# Autodesk Inventor assembly: Сборка4
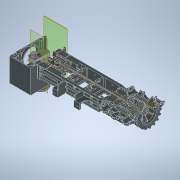
[picture p0: Inventor's stored thumbnail of the model, 180x180]
Saved by Autodesk Inventor 2021 (Build 250183000, 183)
## iProperties
Created: 2020-11-22
Part Number: Сборка4
Document SubType Name: Assembly
Designer: Тимоха
Author: Тимоха
## Documents named in this file (66)
- C:\Users\Тимоха\Desktop\КР Компрессор\compressor\Сборка4.iam
- C:\Users\Тимоха\Desktop\КР Компрессор\compressor\Верхняя часть поршня.ipt
- C:\Users\Тимоха\Desktop\КР Компрессор\compressor\Втулка.ipt
- C:\Users\Тимоха\Desktop\КР Компрессор\compressor\Гайка шток-поршень.ipt
- C:\Users\Тимоха\Desktop\КР Компрессор\compressor\Дроссельное кольцо.ipt
- C:\Users\Тимоха\Desktop\КР Компрессор\compressor\Клапан1.iam
- C:\Users\Тимоха\Desktop\КР Компрессор\compressor\Кольцо поршень-шток верх.ipt
- C:\Users\Тимоха\Desktop\КР Компрессор\compressor\Кольцо поршень-шток низ.ipt
- C:\Users\Тимоха\Desktop\КР Компрессор\compressor\Кольцо поршня.ipt
- C:\Users\Тимоха\Desktop\КР Компрессор\compressor\Кольцо сальника.ipt
- C:\Users\Тимоха\Desktop\КР Компрессор\compressor\Корпус дросселя.ipt
- C:\Users\Тимоха\Desktop\КР Компрессор\compressor\Корпус сальника.ipt
- C:\Users\Тимоха\Desktop\КР Компрессор\compressor\Крышка сальников.ipt
- C:\Users\Тимоха\Desktop\КР Компрессор\compressor\Крышка стакана.ipt
- C:\Users\Тимоха\Desktop\КР Компрессор\compressor\Крышка цилиндра 1.ipt
- C:\Users\Тимоха\Desktop\КР Компрессор\compressor\Крышка цилиндра 2.ipt
- C:\Users\Тимоха\Desktop\КР Компрессор\compressor\Нижняя часть поршня.ipt
- C:\Users\Тимоха\Desktop\КР Компрессор\compressor\Опорное кольцо.ipt
- C:\Users\Тимоха\Desktop\КР Компрессор\compressor\Прокладка клапана.ipt
- C:\Users\Тимоха\Desktop\КР Компрессор\compressor\Пружина дросселя.ipt
- C:\Users\Тимоха\Desktop\КР Компрессор\compressor\Пружина сальника.ipt
- C:\Users\Тимоха\Desktop\КР Компрессор\compressor\Стакан1.ipt
- C:\Users\Тимоха\Desktop\КР Компрессор\compressor\Цилиндр2.ipt
- C:\Users\Тимоха\Desktop\КР Компрессор\compressor\Шток.ipt
- C:\Users\Тимоха\Documents\Inventor\Content Center Files\R2021\ru-RU\Stud GOST 22034-76\Шпилька M20-6g×50 ГОСТ 22034-76.ipt
- C:\Users\Тимоха\Documents\Inventor\Content Center Files\R2021\ru-RU\GOST 10450-78\Шайба 21 ГОСТ 10450-78.ipt
- C:\Users\Тимоха\Documents\Inventor\Content Center Files\R2021\ru-RU\GOST 15521-70\Гайка M20-6H ГОСТ 15521-70.ipt
- C:\Users\Тимоха\Documents\Inventor\Content Center Files\R2021\ru-RU\GOST 11371-78  A\Шайба 24 ГОСТ 11371-78.ipt
- C:\Users\Тимоха\Documents\Inventor\Content Center Files\R2021\ru-RU\Stud GOST 22038-76\Шпилька M24-6g×70 ГОСТ 22038-76.ipt
- C:\Users\Тимоха\Documents\Inventor\Content Center Files\R2021\ru-RU\Nut GOST 15524-70\Гайка M24-6H ГОСТ 15524-70.ipt
- C:\Users\Тимоха\Documents\Inventor\Content Center Files\R2021\ru-RU\Bolt GOST R 50274-92\Болт M8-6g×20-F ГОСТ Р 50274-92.ipt
- C:\Users\Тимоха\Desktop\КР Компрессор\compressor\Деталь5.ipt
- C:\Users\Тимоха\Desktop\КР Компрессор\compressor\Деталь6.ipt
- C:\Users\Тимоха\Desktop\КР Компрессор\compressor\Прокладка воды зад.ipt
- C:\Users\Тимоха\Desktop\КР Компрессор\compressor\Крышка воды зад.ipt
- C:\Users\Тимоха\Documents\Inventor\Content Center Files\R2021\ru-RU\GOST 15521-70\Гайка M10-6H ГОСТ 15521-70.ipt
- C:\Users\Тимоха\Documents\Inventor\Content Center Files\R2021\ru-RU\Stud GOST 22034-76\Шпилька M10-6g×45 ГОСТ 22034-76.ipt
- C:\Users\Тимоха\Documents\Inventor\Content Center Files\R2021\ru-RU\Washer GOST 9065-75\Шайба 12 ГОСТ 9065-75.ipt
- C:\Users\Тимоха\Desktop\КР Компрессор\compressor\Фонарь.ipt
- C:\Users\Тимоха\Documents\Inventor\Content Center Files\R2021\ru-RU\Stud GOST 22038-76\Шпилька M20-6g×80 ГОСТ 22038-76.ipt
- C:\Users\Тимоха\Documents\Inventor\Content Center Files\R2021\ru-RU\GOST 6402-70\Шайба  22 L ГОСТ 6402-70.ipt
- C:\Users\Тимоха\Documents\Inventor\Content Center Files\R2021\ru-RU\Nut GOST ISO 8673-2014\Копия Копия гайки M20x1,5-6H ГОСТ 5915-70.ipt
- C:\Users\Тимоха\Desktop\КР Компрессор\compressor\Корпус сальника перегородка 1.ipt
- C:\Users\Тимоха\Desktop\КР Компрессор\compressor\Крышка перегородки11.ipt
- C:\Users\Тимоха\Desktop\КР Компрессор\compressor\Крышка перегородки12.ipt
- C:\Users\Тимоха\Desktop\КР Компрессор\compressor\Придав перегородки1.ipt
- C:\Users\Тимоха\Desktop\КР Компрессор\compressor\Корпус маслосъемника.ipt
- C:\Users\Тимоха\Desktop\КР Компрессор\compressor\Крышка перегородки21.ipt
- C:\Users\Тимоха\Desktop\КР Компрессор\compressor\Крышка перегородки22.ipt
- C:\Users\Тимоха\Desktop\КР Компрессор\compressor\Маслосъемная пружина.ipt
- C:\Users\Тимоха\Desktop\КР Компрессор\compressor\Маслосъемное кольцо.ipt
- C:\Users\Тимоха\Documents\Inventor\Content Center Files\R2021\ru-RU\GOST 11738-84\Винт M10-6gx20 ГОСТ 11738-84.ipt
- C:\Users\Тимоха\Documents\Inventor\Content Center Files\R2021\ru-RU\GOST 11371-78  A\Шайба 12 ГОСТ 11371-78.ipt
- C:\Users\Тимоха\Documents\Inventor\Content Center Files\R2021\ru-RU\GOST 11738-84\Винт M10-6gx25 ГОСТ 11738-84.ipt
- C:\Users\Тимоха\Desktop\КР Компрессор\compressor\Крейцкопфф.iam
- C:\Users\Тимоха\Desktop\КР Компрессор\compressor\Вал.ipt
- C:\Users\Тимоха\Desktop\КР Компрессор\compressor\Крышка фонаря 1.ipt
- C:\Users\Тимоха\Desktop\КР Компрессор\compressor\Крышка фонаря 2.ipt
- C:\Users\Тимоха\Desktop\КР Компрессор\compressor\Крышка коренного подшипника1.ipt
- C:\Users\Тимоха\Desktop\КР Компрессор\compressor\Картер.ipt
- C:\Users\Тимоха\Desktop\КР Компрессор\compressor\Балка.ipt
- C:\Users\Тимоха\Desktop\КР Компрессор\compressor\Крышка стенки картера низ.ipt
- C:\Users\Тимоха\Desktop\КР Компрессор\compressor\Нижняя часть коренного подшипника.ipt
- C:\Users\Тимоха\Desktop\КР Компрессор\compressor\Крышка стенки картера верх.ipt
- C:\Users\Тимоха\Desktop\КР Компрессор\compressor\Крышка картера 1.ipt
- C:\Users\Тимоха\Desktop\КР Компрессор\compressor\Крышка картера 3.ipt
## Components (455 placed, 65 different names)
1. Втулка:1 — Жесткий:9, Жесткий:12
2. Дроссельное кольцо:1 — Жесткий:21, Жесткий:22
3. Клапан1:1 [sub-assembly] — Жесткий:11, С поворотом:4
4. Корпус дросселя:1 — Жесткий:22, С поворотом:6
5. Крышка сальников:1 — Жесткий:72, Жесткий:73, Жесткий:143
6. Крышка стакана:1 — С поворотом:5
7. Крышка цилиндра 1:1 — Жесткий:12, С поворотом:9, Жесткий:198, Угол:1, Угол:2, Угол:3
8. Крышка цилиндра 2:1 — Жесткий:13, С поворотом:6, Жесткий:79, Жесткий:142, Жесткий:145, С поворотом:16
9. Прокладка клапана:1 — Жесткий:10, Жесткий:11
10. Пружина дросселя:1 — Жесткий:21
11. Стакан1:1 — С поворотом:4, С поворотом:5
12. Цилиндр2:1 — Жесткий:9, Жесткий:10, Жесткий:13, Жесткий:74, Жесткий:76, Жесткий:80, Заподлицо:1, Заподлицо:2, Заподлицо:5, Заподлицо:6
13. Кольцо сальника:4
14. Корпус сальника:2 — Жесткий:65
15. Пружина сальника:4
16. Кольцо сальника:5
17. Пружина сальника:5
18. Кольцо сальника:6
19. Пружина сальника:6
20. Кольцо сальника:7
21. Корпус сальника:3 — Жесткий:69, Жесткий:73
22. Пружина сальника:7
23. Кольцо сальника:8
24. Пружина сальника:8
25. Кольцо сальника:9
26. Пружина сальника:9
27. Кольцо сальника:10
28. Корпус сальника:4 — Жесткий:66
29. Пружина сальника:10
30. Кольцо сальника:11
31. Пружина сальника:11
32. Кольцо сальника:12
33. Пружина сальника:12
34. Кольцо сальника:13
35. Корпус сальника:5 — Жесткий:68
36. Пружина сальника:13
37. Кольцо сальника:14
38. Пружина сальника:14
39. Кольцо сальника:15
40. Пружина сальника:15
41. Кольцо сальника:16
42. Корпус сальника:6 — Жесткий:68, Жесткий:69
43. Пружина сальника:16
44. Кольцо сальника:17
45. Пружина сальника:17
46. Кольцо сальника:18
47. Пружина сальника:18
48. Кольцо сальника:19
49. Корпус сальника:7 — Жесткий:65, Жесткий:66
50. Пружина сальника:19
51. Кольцо сальника:20
52. Пружина сальника:20
53. Кольцо сальника:21
54. Пружина сальника:21
55. Кольцо сальника:22 — Жесткий:70, Жесткий:140
56. Кольцо сальника:23 — Жесткий:70, Жесткий:71, Жесткий:139
57. Кольцо сальника:24 — Жесткий:71, Жесткий:72, Жесткий:141
58. Болт ГОСТ Р 50274-92 M8-6g×20-F:2 — Жесткий:82
59. Болт ГОСТ Р 50274-92 M8-6g×20-F:3 — Жесткий:81
60. Деталь5:1 — Заподлицо:1, Заподлицо:2, Заподлицо:3, Заподлицо:4
61. Деталь6:1 — Заподлицо:3, Заподлицо:4, Жесткий:81, Жесткий:82, С поворотом:10, С поворотом:11, С поворотом:12, С поворотом:13, С поворотом:14, Жесткий:83, Жесткий:84, Жесткий:85, Жесткий:86, Жесткий:87, Жесткий:88, Жесткий:89, Жесткий:90, Жесткий:91, Жесткий:92, Жесткий:93, Жесткий:94, Жесткий:95, Жесткий:96, Жесткий:97, Жесткий:98, Жесткий:99, Жесткий:100, Жесткий:101, Жесткий:102, Жесткий:103, Жесткий:104, Жесткий:105, Жесткий:106, Жесткий:107
62. Прокладка воды зад:1 — Заподлицо:5, Заподлицо:6, Заподлицо:7, Заподлицо:8
63. Крышка воды зад:1 — Заподлицо:7, Заподлицо:8, С поворотом:15, Жесткий:108, Жесткий:109, Жесткий:110, Жесткий:111, Жесткий:112, Жесткий:113, Жесткий:114, Жесткий:115, Жесткий:116, Жесткий:117, Жесткий:118, Жесткий:119, Жесткий:120, Жесткий:121, Жесткий:122, Жесткий:123, Жесткий:124, Жесткий:125, Жесткий:126, Жесткий:127, Жесткий:128, Жесткий:129, Жесткий:130, Жесткий:131, Жесткий:132, Жесткий:133, Жесткий:134, Жесткий:135, Жесткий:136, Жесткий:137, Жесткий:138
64. Болт ГОСТ Р 50274-92 M8-6g×20-F:33 — С поворотом:14
65. Болт ГОСТ Р 50274-92 M8-6g×20-F:34 — Жесткий:85
66. Болт ГОСТ Р 50274-92 M8-6g×20-F:35 — С поворотом:11
67. Болт ГОСТ Р 50274-92 M8-6g×20-F:36 — С поворотом:10
68. Болт ГОСТ Р 50274-92 M8-6g×20-F:37 — Жесткий:83
69. Болт ГОСТ Р 50274-92 M8-6g×20-F:38 — Жесткий:84
70. Болт ГОСТ Р 50274-92 M8-6g×20-F:39 — С поворотом:12
71. Болт ГОСТ Р 50274-92 M8-6g×20-F:40 — С поворотом:13
72. Болт ГОСТ Р 50274-92 M8-6g×20-F:41 — Жесткий:91
73. Болт ГОСТ Р 50274-92 M8-6g×20-F:42 — Жесткий:90
74. Болт ГОСТ Р 50274-92 M8-6g×20-F:43 — Жесткий:87
75. Болт ГОСТ Р 50274-92 M8-6g×20-F:44 — Жесткий:86
76. Болт ГОСТ Р 50274-92 M8-6g×20-F:45 — Жесткий:89
77. Болт ГОСТ Р 50274-92 M8-6g×20-F:46 — Жесткий:93
78. Болт ГОСТ Р 50274-92 M8-6g×20-F:47 — Жесткий:88
79. Болт ГОСТ Р 50274-92 M8-6g×20-F:48 — Жесткий:92
80. Болт ГОСТ Р 50274-92 M8-6g×20-F:49 — Жесткий:99
81. Болт ГОСТ Р 50274-92 M8-6g×20-F:50 — Жесткий:98
82. Болт ГОСТ Р 50274-92 M8-6g×20-F:51 — Жесткий:97
83. Болт ГОСТ Р 50274-92 M8-6g×20-F:52 — Жесткий:94
84. Болт ГОСТ Р 50274-92 M8-6g×20-F:53 — Жесткий:95
85. Болт ГОСТ Р 50274-92 M8-6g×20-F:54 — Жесткий:102
86. Болт ГОСТ Р 50274-92 M8-6g×20-F:55 — Жесткий:100
87. Болт ГОСТ Р 50274-92 M8-6g×20-F:56 — Жесткий:101
88. Болт ГОСТ Р 50274-92 M8-6g×20-F:58 — Жесткий:106
89. Болт ГОСТ Р 50274-92 M8-6g×20-F:59 — Жесткий:104
90. Болт ГОСТ Р 50274-92 M8-6g×20-F:60 — Жесткий:96
91. Болт ГОСТ Р 50274-92 M8-6g×20-F:61 — Жесткий:107
92. Болт ГОСТ Р 50274-92 M8-6g×20-F:63 — Жесткий:103
93. Болт ГОСТ Р 50274-92 M8-6g×20-F:64 — Жесткий:105
94. Болт ГОСТ Р 50274-92 M8-6g×20-F:68 — С поворотом:15
95. Болт ГОСТ Р 50274-92 M8-6g×20-F:97 — Жесткий:108
96. Болт ГОСТ Р 50274-92 M8-6g×20-F:98 — Жесткий:110
97. Болт ГОСТ Р 50274-92 M8-6g×20-F:99 — Жесткий:109
98. Болт ГОСТ Р 50274-92 M8-6g×20-F:100 — Жесткий:111
99. Болт ГОСТ Р 50274-92 M8-6g×20-F:101 — Жесткий:113
100. Болт ГОСТ Р 50274-92 M8-6g×20-F:102 — Жесткий:112
101. Болт ГОСТ Р 50274-92 M8-6g×20-F:103 — Жесткий:114
102. Болт ГОСТ Р 50274-92 M8-6g×20-F:104 — Жесткий:115
103. Болт ГОСТ Р 50274-92 M8-6g×20-F:105 — Жесткий:116
104. Болт ГОСТ Р 50274-92 M8-6g×20-F:106 — Жесткий:118
105. Болт ГОСТ Р 50274-92 M8-6g×20-F:107 — Жесткий:130
106. Болт ГОСТ Р 50274-92 M8-6g×20-F:108 — Жесткий:134
107. Болт ГОСТ Р 50274-92 M8-6g×20-F:109 — Жесткий:133
108. Болт ГОСТ Р 50274-92 M8-6g×20-F:110 — Жесткий:131
109. Болт ГОСТ Р 50274-92 M8-6g×20-F:111 — Жесткий:135
110. Болт ГОСТ Р 50274-92 M8-6g×20-F:112 — Жесткий:132
111. Болт ГОСТ Р 50274-92 M8-6g×20-F:117 — Жесткий:117
112. Болт ГОСТ Р 50274-92 M8-6g×20-F:118 — Жесткий:119
113. Болт ГОСТ Р 50274-92 M8-6g×20-F:119 — Жесткий:120
114. Болт ГОСТ Р 50274-92 M8-6g×20-F:120 — Жесткий:121
115. Болт ГОСТ Р 50274-92 M8-6g×20-F:121 — Жесткий:122
116. Болт ГОСТ Р 50274-92 M8-6g×20-F:122 — Жесткий:123
117. Болт ГОСТ Р 50274-92 M8-6g×20-F:123 — Жесткий:124
118. Болт ГОСТ Р 50274-92 M8-6g×20-F:124 — Жесткий:125
119. Болт ГОСТ Р 50274-92 M8-6g×20-F:125 — Жесткий:126
120. Болт ГОСТ Р 50274-92 M8-6g×20-F:126 — Жесткий:127
121. Болт ГОСТ Р 50274-92 M8-6g×20-F:130 — Жесткий:129
122. Болт ГОСТ Р 50274-92 M8-6g×20-F:137 — Жесткий:128
123. Болт ГОСТ Р 50274-92 M8-6g×20-F:138 — Жесткий:137
124. Болт ГОСТ Р 50274-92 M8-6g×20-F:139 — Жесткий:136
125. Болт ГОСТ Р 50274-92 M8-6g×20-F:140 — Жесткий:138
126. Пружина сальника:22 — Жесткий:141
127. Пружина сальника:23 — Жесткий:140
128. Пружина сальника:24 — Жесткий:139
129. Фонарь:1 — Жесткий:145, Жесткий:146, Жесткий:160, Жесткий:168, Жесткий:189, Заподлицо:9, Заподлицо:10, Заподлицо:11, Заподлицо:12, Жесткий:211
130. Кольцо сальника:25 — Жесткий:148, Жесткий:152
131. Корпус сальника перегородка 1:1 — Жесткий:158, Жесткий:159, Жесткий:161, Жесткий:162
132. Крышка перегородки11:1 — Жесткий:160, Жесткий:161, Жесткий:163
133. Крышка перегородки12:1 — Жесткий:162, Жесткий:188
134. Придав перегородки1:1 — Жесткий:163, Жесткий:184
135. Пружина сальника:25 — Жесткий:148
136. Кольцо сальника:26 — Жесткий:151, Жесткий:158
137. Пружина сальника:26
138. Кольцо сальника:27 — Жесткий:151, Жесткий:152
139. Пружина сальника:27
140. Кольцо сальника:28 — Жесткий:159
141. Пружина сальника:28
142. Кольцо сальника:29
143. Пружина сальника:29
144. Кольцо сальника:30
145. Пружина сальника:30
146. Корпус маслосъемника:1 — Жесткий:167, Жесткий:175
147. Крышка перегородки21:1 — Жесткий:168, Жесткий:174, Жесткий:175, Жесткий:176, Жесткий:179
148. Крышка перегородки22:1 — Жесткий:176, Жесткий:185
149. Маслосъемное кольцо:1 — Жесткий:166, Жесткий:177
150. Придав перегородки1:2 — Жесткий:179, Жесткий:180
151. Маслосъемное кольцо:2 — Жесткий:166, Жесткий:167, Жесткий:178
152. Кольцо сальника:31 — Жесткий:174
153. Пружина сальника:31
154. Кольцо сальника:32
155. Пружина сальника:32
156. Кольцо сальника:33
157. Пружина сальника:33
158. Маслосъемная пружина:3 — Жесткий:177
159. Маслосъемная пружина:4 — Жесткий:178
160. Крейцкопфф:1 [sub-assembly] — Жесткий:189, Угол:1, Угол:2, Угол:3, С поворотом:19, Угол:4
161. Верхняя часть поршня:2 — Жесткий:198
162. Кольцо поршень-шток низ:2
163. Кольцо поршня:4
164. Нижняя часть поршня:2
165. Опорное кольцо:3
166. Кольцо поршня:5
167. Кольцо поршня:6
168. Опорное кольцо:4
169. Гайка шток-поршень:2
170. Кольцо поршень-шток верх:2
171. Шток:2
172. Вал:1 — С поворотом:19, Угол:4, Цилиндрический:1, Совмещение:1
173. Крышка фонаря 1:1 — Заподлицо:9, Заподлицо:10
174. Крышка фонаря 2:1 — Заподлицо:11, Заподлицо:12
175. Картер:1 — Жесткий:211
176. Балка:1
177. Балка:2
178. Крышка стенки картера низ:1
179. Нижняя часть коренного подшипника:1 — Цилиндрический:1
180. Нижняя часть коренного подшипника:2
181. Нижняя часть коренного подшипника:3
182. Крышка стенки картера верх:1
183. Крышка коренного подшипника1:1
184. Нижняя часть коренного подшипника:4
185. Крышка картера 1:1
186. Крышка картера 3:1
187. Крышка коренного подшипника1:2 — Совмещение:1
188. Гайка ГОСТ 15524-70 M24:1 — Жесткий:77
189. Шайба  ГОСТ 11371-78 25:1 — Жесткий:77, С поворотом:9
190. Шпилька ГОСТ 22038-76 M24-6g×70:1 — Жесткий:76
191. Гайка ГОСТ 15524-70 M24:2
192. Шайба  ГОСТ 11371-78 25:2
193. Шпилька ГОСТ 22038-76 M24-6g×70:2
194. Гайка ГОСТ 15524-70 M24:3
195. Шайба  ГОСТ 11371-78 25:3
196. Шпилька ГОСТ 22038-76 M24-6g×70:3
197. Гайка ГОСТ 15524-70 M24:4
198. Шайба  ГОСТ 11371-78 25:4
199. Шпилька ГОСТ 22038-76 M24-6g×70:4
200. Гайка ГОСТ 15524-70 M24:5
201. Шайба  ГОСТ 11371-78 25:5
202. Шпилька ГОСТ 22038-76 M24-6g×70:5
203. Гайка ГОСТ 15524-70 M24:6
204. Шайба  ГОСТ 11371-78 25:6
205. Шпилька ГОСТ 22038-76 M24-6g×70:6
206. Гайка ГОСТ 15524-70 M24:7
207. Шайба  ГОСТ 11371-78 25:7
208. Шпилька ГОСТ 22038-76 M24-6g×70:7
209. Гайка ГОСТ 15524-70 M24:8
210. Шайба  ГОСТ 11371-78 25:8
211. Шпилька ГОСТ 22038-76 M24-6g×70:8
212. Гайка ГОСТ 15524-70 M24:9
213. Шайба  ГОСТ 11371-78 25:9
214. Шпилька ГОСТ 22038-76 M24-6g×70:9
215. Гайка ГОСТ 15524-70 M24:10
216. Шайба  ГОСТ 11371-78 25:10
217. Шпилька ГОСТ 22038-76 M24-6g×70:10
218. Гайка ГОСТ 15524-70 M24:11
219. Шайба  ГОСТ 11371-78 25:11
220. Шпилька ГОСТ 22038-76 M24-6g×70:11
221. Гайка ГОСТ 15524-70 M24:12
222. Шайба  ГОСТ 11371-78 25:12
223. Шпилька ГОСТ 22038-76 M24-6g×70:12
224. Гайка ГОСТ 15524-70 M24:13
225. Шайба  ГОСТ 11371-78 25:13
226. Шпилька ГОСТ 22038-76 M24-6g×70:13
227. Гайка ГОСТ 15524-70 M24:14
228. Шайба  ГОСТ 11371-78 25:14
229. Шпилька ГОСТ 22038-76 M24-6g×70:14
230. Гайка ГОСТ 15524-70 M24:15
231. Шайба  ГОСТ 11371-78 25:15
232. Шпилька ГОСТ 22038-76 M24-6g×70:15
233. Гайка ГОСТ 15524-70 M24:16
234. Шайба  ГОСТ 11371-78 25:16
235. Шпилька ГОСТ 22038-76 M24-6g×70:16
236. Шпилька ГОСТ 22038-76 M24-6g×70:17 — Жесткий:80
237. Гайка ГОСТ 15524-70 M24:17
238. Шайба  ГОСТ 11371-78 25:17 — Жесткий:79
239. Шпилька ГОСТ 22038-76 M24-6g×70:18
240. Гайка ГОСТ 15524-70 M24:18
241. Шайба  ГОСТ 11371-78 25:18
242. Шпилька ГОСТ 22038-76 M24-6g×70:19
243. Гайка ГОСТ 15524-70 M24:19
244. Шайба  ГОСТ 11371-78 25:19
245. Шпилька ГОСТ 22038-76 M24-6g×70:20
246. Гайка ГОСТ 15524-70 M24:20
247. Шайба  ГОСТ 11371-78 25:20
248. Шпилька ГОСТ 22038-76 M24-6g×70:21
249. Гайка ГОСТ 15524-70 M24:21
250. Шайба  ГОСТ 11371-78 25:21
251. Шпилька ГОСТ 22038-76 M24-6g×70:22
252. Гайка ГОСТ 15524-70 M24:22
253. Шайба  ГОСТ 11371-78 25:22
254. Шпилька ГОСТ 22038-76 M24-6g×70:23
255. Гайка ГОСТ 15524-70 M24:23
256. Шайба  ГОСТ 11371-78 25:23
257. Шпилька ГОСТ 22038-76 M24-6g×70:24
258. Гайка ГОСТ 15524-70 M24:24
259. Шайба  ГОСТ 11371-78 25:24
260. Шпилька ГОСТ 22038-76 M24-6g×70:25
261. Гайка ГОСТ 15524-70 M24:25
262. Шайба  ГОСТ 11371-78 25:25
263. Шпилька ГОСТ 22038-76 M24-6g×70:26
264. Гайка ГОСТ 15524-70 M24:26
265. Шайба  ГОСТ 11371-78 25:26
266. Шпилька ГОСТ 22038-76 M24-6g×70:27
267. Гайка ГОСТ 15524-70 M24:27
268. Шайба  ГОСТ 11371-78 25:27
269. Шпилька ГОСТ 22038-76 M24-6g×70:28
270. Гайка ГОСТ 15524-70 M24:28
271. Шайба  ГОСТ 11371-78 25:28
272. Шпилька ГОСТ 22038-76 M24-6g×70:29
273. Гайка ГОСТ 15524-70 M24:29
274. Шайба  ГОСТ 11371-78 25:29
275. Шпилька ГОСТ 22038-76 M24-6g×70:30
276. Гайка ГОСТ 15524-70 M24:30
277. Шайба  ГОСТ 11371-78 25:30
278. Шпилька ГОСТ 22038-76 M24-6g×70:31
279. Гайка ГОСТ 15524-70 M24:31
280. Шайба  ГОСТ 11371-78 25:31
281. Шпилька ГОСТ 22038-76 M24-6g×70:32
282. Гайка ГОСТ 15524-70 M24:32
283. Шайба  ГОСТ 11371-78 25:32
284. Шпилька ГОСТ 22034-76 M10-6g×45:1 — Жесткий:142
285. Гайка ГОСТ 15521-70 M10:1 — Жесткий:144
286. Шайба ГОСТ 9065-75 12:1 — Жесткий:143, Жесткий:144
287. Шпилька ГОСТ 22034-76 M10-6g×45:2
288. Гайка ГОСТ 15521-70 M10:2
289. Шайба ГОСТ 9065-75 12:2
290. Шпилька ГОСТ 22034-76 M10-6g×45:3
291. Гайка ГОСТ 15521-70 M10:3
292. Шайба ГОСТ 9065-75 12:3
293. Шпилька ГОСТ 22034-76 M10-6g×45:4
294. Гайка ГОСТ 15521-70 M10:4
295. Шайба ГОСТ 9065-75 12:4
296. Шпилька ГОСТ 22034-76 M10-6g×45:5
297. Гайка ГОСТ 15521-70 M10:5
298. Шайба ГОСТ 9065-75 12:5
299. Шпилька ГОСТ 22034-76 M10-6g×45:6
300. Гайка ГОСТ 15521-70 M10:6
301. Шайба ГОСТ 9065-75 12:6
302. Шпилька ГОСТ 22034-76 M10-6g×45:7
303. Гайка ГОСТ 15521-70 M10:7
304. Шайба ГОСТ 9065-75 12:7
305. Шпилька ГОСТ 22034-76 M10-6g×45:8
306. Гайка ГОСТ 15521-70 M10:8
307. Шайба ГОСТ 9065-75 12:8
308. Шпилька ГОСТ 22034-76 M10-6g×45:9
309. Гайка ГОСТ 15521-70 M10:9
310. Шайба ГОСТ 9065-75 12:9
311. Шпилька ГОСТ 22034-76 M10-6g×45:10
312. Гайка ГОСТ 15521-70 M10:10
313. Шайба ГОСТ 9065-75 12:10
314. Шпилька ГОСТ 22038-76 M20-6g×80:1 — С поворотом:16
315. Гайка ГОСТ ISO 8673-2014 M20x1,5:1 — Жесткий:147
316. Шайба ГОСТ 6402-70 22 L:1 — Жесткий:146, Жесткий:147
317. Шпилька ГОСТ 22038-76 M20-6g×80:2
318. Гайка ГОСТ ISO 8673-2014 M20x1,5:2
319. Шайба ГОСТ 6402-70 22 L:2
320. Шпилька ГОСТ 22038-76 M20-6g×80:3
321. Гайка ГОСТ ISO 8673-2014 M20x1,5:3
322. Шайба ГОСТ 6402-70 22 L:3
323. Шпилька ГОСТ 22038-76 M20-6g×80:4
324. Гайка ГОСТ ISO 8673-2014 M20x1,5:4
325. Шайба ГОСТ 6402-70 22 L:4
326. Шпилька ГОСТ 22038-76 M20-6g×80:5
327. Гайка ГОСТ ISO 8673-2014 M20x1,5:5
328. Шайба ГОСТ 6402-70 22 L:5
329. Шпилька ГОСТ 22038-76 M20-6g×80:6
330. Гайка ГОСТ ISO 8673-2014 M20x1,5:6
331. Шайба ГОСТ 6402-70 22 L:6
332. Шпилька ГОСТ 22038-76 M20-6g×80:7
333. Гайка ГОСТ ISO 8673-2014 M20x1,5:7
334. Шайба ГОСТ 6402-70 22 L:7
335. Шпилька ГОСТ 22038-76 M20-6g×80:8
336. Гайка ГОСТ ISO 8673-2014 M20x1,5:8
337. Шайба ГОСТ 6402-70 22 L:8
338. Шпилька ГОСТ 22038-76 M20-6g×80:9
339. Гайка ГОСТ ISO 8673-2014 M20x1,5:9
340. Шайба ГОСТ 6402-70 22 L:9
341. Шпилька ГОСТ 22038-76 M20-6g×80:10
342. Гайка ГОСТ ISO 8673-2014 M20x1,5:10
343. Шайба ГОСТ 6402-70 22 L:10
344. Шпилька ГОСТ 22038-76 M20-6g×80:11
345. Гайка ГОСТ ISO 8673-2014 M20x1,5:11
346. Шайба ГОСТ 6402-70 22 L:11
347. Шпилька ГОСТ 22038-76 M20-6g×80:12
348. Гайка ГОСТ ISO 8673-2014 M20x1,5:12
349. Шайба ГОСТ 6402-70 22 L:12
350. Шпилька ГОСТ 22038-76 M20-6g×80:13
351. Гайка ГОСТ ISO 8673-2014 M20x1,5:13
352. Шайба ГОСТ 6402-70 22 L:13
353. Шпилька ГОСТ 22038-76 M20-6g×80:14
354. Гайка ГОСТ ISO 8673-2014 M20x1,5:14
355. Шайба ГОСТ 6402-70 22 L:14
356. Шпилька ГОСТ 22038-76 M20-6g×80:15
357. Гайка ГОСТ ISO 8673-2014 M20x1,5:15
358. Шайба ГОСТ 6402-70 22 L:15
359. Шпилька ГОСТ 22038-76 M20-6g×80:16
360. Гайка ГОСТ ISO 8673-2014 M20x1,5:16
361. Шайба ГОСТ 6402-70 22 L:16
362. Гайка ГОСТ 15521-70 M20:1 — Жесткий:75
363. Шпилька ГОСТ 22034-76 M20-6g×50:1 — Жесткий:74, Жесткий:75
364. Шайба ГОСТ 10450-78 21:1
365. Гайка ГОСТ 15521-70 M20:2
366. Шпилька ГОСТ 22034-76 M20-6g×50:2
367. Шайба ГОСТ 10450-78 21:2
368. Гайка ГОСТ 15521-70 M20:3
369. Шпилька ГОСТ 22034-76 M20-6g×50:3
370. Шайба ГОСТ 10450-78 21:3
371. Гайка ГОСТ 15521-70 M20:4
372. Шпилька ГОСТ 22034-76 M20-6g×50:4
373. Шайба ГОСТ 10450-78 21:4
374. Гайка ГОСТ 15521-70 M20:5
375. Шпилька ГОСТ 22034-76 M20-6g×50:5
376. Шайба ГОСТ 10450-78 21:5
377. Гайка ГОСТ 15521-70 M20:6
378. Шпилька ГОСТ 22034-76 M20-6g×50:6
379. Шайба ГОСТ 10450-78 21:6
380. Гайка ГОСТ 15521-70 M20:7
381. Шпилька ГОСТ 22034-76 M20-6g×50:7
382. Шайба ГОСТ 10450-78 21:7
383. Гайка ГОСТ 15521-70 M20:8
384. Шпилька ГОСТ 22034-76 M20-6g×50:8
385. Шайба ГОСТ 10450-78 21:8
386. Гайка ГОСТ 15521-70 M20:9
387. Шпилька ГОСТ 22034-76 M20-6g×50:9
388. Шайба ГОСТ 10450-78 21:9
389. Гайка ГОСТ 15521-70 M20:10
390. Шпилька ГОСТ 22034-76 M20-6g×50:10
391. Шайба ГОСТ 10450-78 21:10
392. Винт ГОСТ 11738-84 M 10x20:1 — Жесткий:181
393. Шайба  ГОСТ 11371-78 13:1 — Жесткий:180, Жесткий:181
394. Винт ГОСТ 11738-84 M 10x20:4
395. Шайба  ГОСТ 11371-78 13:4
396. Винт ГОСТ 11738-84 M 10x20:5
397. Шайба  ГОСТ 11371-78 13:5
398. Винт ГОСТ 11738-84 M 10x20:6
399. Шайба  ГОСТ 11371-78 13:6
400. Винт ГОСТ 11738-84 M 10x20:7
401. Шайба  ГОСТ 11371-78 13:7
402. Винт ГОСТ 11738-84 M 10x20:8
403. Шайба  ГОСТ 11371-78 13:8
404. Винт ГОСТ 11738-84 M 10x20:9
405. Шайба  ГОСТ 11371-78 13:9
406. Винт ГОСТ 11738-84 M 10x20:10
407. Шайба  ГОСТ 11371-78 13:10
408. Винт ГОСТ 11738-84 M 10x20:3
409. Шайба  ГОСТ 11371-78 13:3 — Жесткий:184
410. Винт ГОСТ 11738-84 M 10x20:11
411. Шайба  ГОСТ 11371-78 13:11
412. Винт ГОСТ 11738-84 M 10x20:12
413. Шайба  ГОСТ 11371-78 13:12
414. Винт ГОСТ 11738-84 M 10x20:13
415. Шайба  ГОСТ 11371-78 13:13
416. Винт ГОСТ 11738-84 M 10x20:14
417. Шайба  ГОСТ 11371-78 13:14
418. Винт ГОСТ 11738-84 M 10x20:15
419. Шайба  ГОСТ 11371-78 13:15
420. Винт ГОСТ 11738-84 M 10x20:16
421. Шайба  ГОСТ 11371-78 13:16
422. Винт ГОСТ 11738-84 M 10x20:17
423. Шайба  ГОСТ 11371-78 13:17
424. Винт ГОСТ 11738-84 M 10x25:2
425. Шайба  ГОСТ 11371-78 13:19 — Жесткий:188
426. Винт ГОСТ 11738-84 M 10x25:3
427. Шайба  ГОСТ 11371-78 13:20
428. Винт ГОСТ 11738-84 M 10x25:4
429. Шайба  ГОСТ 11371-78 13:21
430. Винт ГОСТ 11738-84 M 10x25:5
431. Шайба  ГОСТ 11371-78 13:22
432. Винт ГОСТ 11738-84 M 10x25:6
433. Шайба  ГОСТ 11371-78 13:23
434. Винт ГОСТ 11738-84 M 10x25:7
435. Шайба  ГОСТ 11371-78 13:24
436. Винт ГОСТ 11738-84 M 10x25:8
437. Шайба  ГОСТ 11371-78 13:25
438. Винт ГОСТ 11738-84 M 10x25:9
439. Шайба  ГОСТ 11371-78 13:26
440. Шайба  ГОСТ 11371-78 13:18 — Жесткий:185, Жесткий:186
441. Винт ГОСТ 11738-84 M 10x25:1 — Жесткий:186
442. Шайба  ГОСТ 11371-78 13:27
443. Винт ГОСТ 11738-84 M 10x25:10
444. Шайба  ГОСТ 11371-78 13:28
445. Винт ГОСТ 11738-84 M 10x25:11
446. Шайба  ГОСТ 11371-78 13:29
447. Винт ГОСТ 11738-84 M 10x25:12
448. Шайба  ГОСТ 11371-78 13:30
449. Винт ГОСТ 11738-84 M 10x25:13
450. Шайба  ГОСТ 11371-78 13:31
451. Винт ГОСТ 11738-84 M 10x25:14
452. Шайба  ГОСТ 11371-78 13:32
453. Винт ГОСТ 11738-84 M 10x25:15
454. Шайба  ГОСТ 11371-78 13:33
455. Винт ГОСТ 11738-84 M 10x25:16
## Component patterns: (16 elements, first: Гайка ГОСТ 15524-70 M24:1 + Шайба  ГОСТ 11371-78 25:1 + Шпилька ГОСТ 22038-76 M24-6g×70:1), (16 elements, first: Шпилька ГОСТ 22038-76 M24-6g×70:17 + Гайка ГОСТ 15524-70 M24:17 + Шайба  ГОСТ 11371-78 25:17), (10 elements, first: Шпилька ГОСТ 22034-76 M10-6g×45:1 + Гайка ГОСТ 15521-70 M10:1 + Шайба ГОСТ 9065-75 12:1), (16 elements, first: Шпилька ГОСТ 22038-76 M20-6g×80:1 + Гайка ГОСТ ISO 8673-2014 M20x1,5:1 + Шайба ГОСТ 6402-70 22 L:1), (10 elements, first: Гайка ГОСТ 15521-70 M20:1 + Шпилька ГОСТ 22034-76 M20-6g×50:1 + Шайба ГОСТ 10450-78 21:1), (8 elements, first: Винт ГОСТ 11738-84 M 10x20:1 + Шайба  ГОСТ 11371-78 13:1), (8 elements, first: Винт ГОСТ 11738-84 M 10x20:3 + Шайба  ГОСТ 11371-78 13:3), (8 elements, first: Винт ГОСТ 11738-84 M 10x25:2 + Шайба  ГОСТ 11371-78 13:19), (8 elements, first: Шайба  ГОСТ 11371-78 13:18 + Винт ГОСТ 11738-84 M 10x25:1)
## Relationships (227: WeldJoint 186, Flush 20, RevoluteJoint 15, Angle 4, CylindricalJoint 1, Mate 1)
- Жесткий:9 [WeldJoint]: Втулка:1 ↔ Цилиндр2:1
- Жесткий:10 [WeldJoint]: Прокладка клапана:1 ↔ Цилиндр2:1
- Жесткий:11 [WeldJoint]: Клапан1:1 ↔ Прокладка клапана:1
- С поворотом:4 [RevoluteJoint]: Клапан1:1 ↔ Стакан1:1
- С поворотом:5 [RevoluteJoint]: Крышка стакана:1 ↔ Стакан1:1
- Жесткий:12 [WeldJoint]: Втулка:1 ↔ Крышка цилиндра 1:1
- Жесткий:13 [WeldJoint]: Крышка цилиндра 2:1 ↔ Цилиндр2:1
- Жесткий:21 [WeldJoint] (2 mm): Дроссельное кольцо:1 ↔ Пружина дросселя:1
- Жесткий:22 [WeldJoint]: Дроссельное кольцо:1 ↔ Корпус дросселя:1
- С поворотом:6 [RevoluteJoint]: Корпус дросселя:1 ↔ Крышка цилиндра 2:1
- [WeldJoint] (-1 mm): Кольцо сальника:4 ↔ Пружина сальника:4
- [WeldJoint] (-1 mm): Кольцо сальника:5 ↔ Пружина сальника:5
- [WeldJoint] (-1 mm): Кольцо сальника:6 ↔ Пружина сальника:6
- [WeldJoint]: Кольцо сальника:5 ↔ Кольцо сальника:6
- [WeldJoint]: Кольцо сальника:4 ↔ Кольцо сальника:5
- [WeldJoint]: Корпус сальника:2 ↔ Кольцо сальника:6
- [WeldJoint] (-1 mm): Кольцо сальника:7 ↔ Пружина сальника:7
- [WeldJoint] (-1 mm): Кольцо сальника:8 ↔ Пружина сальника:8
- [WeldJoint] (-1 mm): Кольцо сальника:9 ↔ Пружина сальника:9
- [WeldJoint]: Кольцо сальника:8 ↔ Кольцо сальника:9
- [WeldJoint]: Кольцо сальника:7 ↔ Кольцо сальника:8
- [WeldJoint]: Корпус сальника:3 ↔ Кольцо сальника:9
- [WeldJoint] (-1 mm): Кольцо сальника:10 ↔ Пружина сальника:10
- [WeldJoint] (-1 mm): Кольцо сальника:11 ↔ Пружина сальника:11
- [WeldJoint] (-1 mm): Кольцо сальника:12 ↔ Пружина сальника:12
- [WeldJoint]: Кольцо сальника:11 ↔ Кольцо сальника:12
- [WeldJoint]: Кольцо сальника:10 ↔ Кольцо сальника:11
- [WeldJoint]: Корпус сальника:4 ↔ Кольцо сальника:12
- [WeldJoint] (-1 mm): Кольцо сальника:13 ↔ Пружина сальника:13
- [WeldJoint] (-1 mm): Кольцо сальника:14 ↔ Пружина сальника:14
- [WeldJoint] (-1 mm): Кольцо сальника:15 ↔ Пружина сальника:15
- [WeldJoint]: Кольцо сальника:14 ↔ Кольцо сальника:15
- [WeldJoint]: Кольцо сальника:13 ↔ Кольцо сальника:14
- [WeldJoint]: Корпус сальника:5 ↔ Кольцо сальника:15
- [WeldJoint] (-1 mm): Кольцо сальника:16 ↔ Пружина сальника:16
- [WeldJoint] (-1 mm): Кольцо сальника:17 ↔ Пружина сальника:17
- [WeldJoint] (-1 mm): Кольцо сальника:18 ↔ Пружина сальника:18
- [WeldJoint]: Кольцо сальника:17 ↔ Кольцо сальника:18
- [WeldJoint]: Кольцо сальника:16 ↔ Кольцо сальника:17
- [WeldJoint]: Корпус сальника:6 ↔ Кольцо сальника:18
- [WeldJoint] (-1 mm): Кольцо сальника:19 ↔ Пружина сальника:19
- [WeldJoint] (-1 mm): Кольцо сальника:20 ↔ Пружина сальника:20
- [WeldJoint] (-1 mm): Кольцо сальника:21 ↔ Пружина сальника:21
- [WeldJoint]: Кольцо сальника:20 ↔ Кольцо сальника:21
- [WeldJoint]: Кольцо сальника:19 ↔ Кольцо сальника:20
- [WeldJoint]: Корпус сальника:7 ↔ Кольцо сальника:21
- Жесткий:65 [WeldJoint]: Корпус сальника:2 ↔ Корпус сальника:7
- Жесткий:66 [WeldJoint]: Корпус сальника:4 ↔ Корпус сальника:7
- Жесткий:68 [WeldJoint]: Корпус сальника:5 ↔ Корпус сальника:6
- Жесткий:69 [WeldJoint]: Корпус сальника:3 ↔ Корпус сальника:6
- Жесткий:70 [WeldJoint]: Кольцо сальника:22 ↔ Кольцо сальника:23
- Жесткий:71 [WeldJoint]: Кольцо сальника:23 ↔ Кольцо сальника:24
- Жесткий:72 [WeldJoint]: Крышка сальников:1 ↔ Кольцо сальника:24
- Жесткий:73 [WeldJoint]: Крышка сальников:1 ↔ Корпус сальника:3
- [RevoluteJoint]: Гайка ГОСТ 15521-70 M20:1 ↔ Шайба ГОСТ 10450-78 21:1
- Жесткий:74 [WeldJoint] (23.5 mm): Цилиндр2:1 ↔ Шпилька ГОСТ 22034-76 M20-6g×50:1
- Жесткий:75 [WeldJoint] (-2.75 mm): Гайка ГОСТ 15521-70 M20:1 ↔ Шпилька ГОСТ 22034-76 M20-6g×50:1
- Жесткий:76 [WeldJoint]: Цилиндр2:1 ↔ Шпилька ГОСТ 22038-76 M24-6g×70:1
- Жесткий:77 [WeldJoint]: Гайка ГОСТ 15524-70 M24:1 ↔ Шайба  ГОСТ 11371-78 25:1
- С поворотом:9 [RevoluteJoint]: Крышка цилиндра 1:1 ↔ Шайба  ГОСТ 11371-78 25:1
- [WeldJoint]: Гайка ГОСТ 15524-70 M24:17 ↔ Шайба  ГОСТ 11371-78 25:17
- Жесткий:79 [WeldJoint]: Крышка цилиндра 2:1 ↔ Шайба  ГОСТ 11371-78 25:17
- Жесткий:80 [WeldJoint]: Цилиндр2:1 ↔ Шпилька ГОСТ 22038-76 M24-6g×70:17
- Заподлицо:1 [Flush]: Цилиндр2:1 ↔ Деталь5:1
- Заподлицо:2 [Flush]: Цилиндр2:1 ↔ Деталь5:1
- Заподлицо:3 [Flush]: Деталь5:1 ↔ Деталь6:1
- Заподлицо:4 [Flush]: Деталь5:1 ↔ Деталь6:1
- Заподлицо:5 [Flush]: Цилиндр2:1 ↔ Прокладка воды зад:1
- Заподлицо:6 [Flush]: Цилиндр2:1 ↔ Прокладка воды зад:1
- Заподлицо:7 [Flush]: Прокладка воды зад:1 ↔ Крышка воды зад:1
- Заподлицо:8 [Flush]: Прокладка воды зад:1 ↔ Крышка воды зад:1
- Жесткий:81 [WeldJoint]: Болт ГОСТ Р 50274-92 M8-6g×20-F:3 ↔ Деталь6:1
- Жесткий:82 [WeldJoint]: Болт ГОСТ Р 50274-92 M8-6g×20-F:2 ↔ Деталь6:1
- С поворотом:10 [RevoluteJoint]: Деталь6:1 ↔ Болт ГОСТ Р 50274-92 M8-6g×20-F:36
- С поворотом:11 [RevoluteJoint]: Деталь6:1 ↔ Болт ГОСТ Р 50274-92 M8-6g×20-F:35
- С поворотом:12 [RevoluteJoint]: Деталь6:1 ↔ Болт ГОСТ Р 50274-92 M8-6g×20-F:39
- С поворотом:13 [RevoluteJoint]: Деталь6:1 ↔ Болт ГОСТ Р 50274-92 M8-6g×20-F:40
- С поворотом:14 [RevoluteJoint]: Деталь6:1 ↔ Болт ГОСТ Р 50274-92 M8-6g×20-F:33
- Жесткий:83 [WeldJoint]: Деталь6:1 ↔ Болт ГОСТ Р 50274-92 M8-6g×20-F:37
- Жесткий:84 [WeldJoint]: Деталь6:1 ↔ Болт ГОСТ Р 50274-92 M8-6g×20-F:38
- Жесткий:85 [WeldJoint]: Деталь6:1 ↔ Болт ГОСТ Р 50274-92 M8-6g×20-F:34
- Жесткий:86 [WeldJoint]: Деталь6:1 ↔ Болт ГОСТ Р 50274-92 M8-6g×20-F:44
- Жесткий:87 [WeldJoint]: Деталь6:1 ↔ Болт ГОСТ Р 50274-92 M8-6g×20-F:43
- Жесткий:88 [WeldJoint]: Деталь6:1 ↔ Болт ГОСТ Р 50274-92 M8-6g×20-F:47
- Жесткий:89 [WeldJoint]: Деталь6:1 ↔ Болт ГОСТ Р 50274-92 M8-6g×20-F:45
- Жесткий:90 [WeldJoint]: Деталь6:1 ↔ Болт ГОСТ Р 50274-92 M8-6g×20-F:42
- Жесткий:91 [WeldJoint]: Деталь6:1 ↔ Болт ГОСТ Р 50274-92 M8-6g×20-F:41
- Жесткий:92 [WeldJoint]: Деталь6:1 ↔ Болт ГОСТ Р 50274-92 M8-6g×20-F:48
- Жесткий:93 [WeldJoint]: Деталь6:1 ↔ Болт ГОСТ Р 50274-92 M8-6g×20-F:46
- Жесткий:94 [WeldJoint]: Деталь6:1 ↔ Болт ГОСТ Р 50274-92 M8-6g×20-F:52
- Жесткий:95 [WeldJoint]: Деталь6:1 ↔ Болт ГОСТ Р 50274-92 M8-6g×20-F:53
- Жесткий:96 [WeldJoint]: Деталь6:1 ↔ Болт ГОСТ Р 50274-92 M8-6g×20-F:60
- Жесткий:97 [WeldJoint]: Деталь6:1 ↔ Болт ГОСТ Р 50274-92 M8-6g×20-F:51
- Жесткий:98 [WeldJoint]: Деталь6:1 ↔ Болт ГОСТ Р 50274-92 M8-6g×20-F:50
- Жесткий:99 [WeldJoint]: Деталь6:1 ↔ Болт ГОСТ Р 50274-92 M8-6g×20-F:49
- Жесткий:100 [WeldJoint]: Деталь6:1 ↔ Болт ГОСТ Р 50274-92 M8-6g×20-F:55
- Жесткий:101 [WeldJoint]: Деталь6:1 ↔ Болт ГОСТ Р 50274-92 M8-6g×20-F:56
- Жесткий:102 [WeldJoint]: Деталь6:1 ↔ Болт ГОСТ Р 50274-92 M8-6g×20-F:54
- Жесткий:103 [WeldJoint]: Деталь6:1 ↔ Болт ГОСТ Р 50274-92 M8-6g×20-F:63
- Жесткий:104 [WeldJoint]: Деталь6:1 ↔ Болт ГОСТ Р 50274-92 M8-6g×20-F:59
- Жесткий:105 [WeldJoint]: Деталь6:1 ↔ Болт ГОСТ Р 50274-92 M8-6g×20-F:64
- Жесткий:106 [WeldJoint]: Деталь6:1 ↔ Болт ГОСТ Р 50274-92 M8-6g×20-F:58
- Жесткий:107 [WeldJoint]: Деталь6:1 ↔ Болт ГОСТ Р 50274-92 M8-6g×20-F:61
- С поворотом:15 [RevoluteJoint]: Крышка воды зад:1 ↔ Болт ГОСТ Р 50274-92 M8-6g×20-F:68
- Жесткий:108 [WeldJoint]: Крышка воды зад:1 ↔ Болт ГОСТ Р 50274-92 M8-6g×20-F:97
- Жесткий:109 [WeldJoint]: Крышка воды зад:1 ↔ Болт ГОСТ Р 50274-92 M8-6g×20-F:99
- Жесткий:110 [WeldJoint]: Крышка воды зад:1 ↔ Болт ГОСТ Р 50274-92 M8-6g×20-F:98
- Жесткий:111 [WeldJoint]: Крышка воды зад:1 ↔ Болт ГОСТ Р 50274-92 M8-6g×20-F:100
- Жесткий:112 [WeldJoint]: Крышка воды зад:1 ↔ Болт ГОСТ Р 50274-92 M8-6g×20-F:102
- Жесткий:113 [WeldJoint]: Крышка воды зад:1 ↔ Болт ГОСТ Р 50274-92 M8-6g×20-F:101
- Жесткий:114 [WeldJoint]: Крышка воды зад:1 ↔ Болт ГОСТ Р 50274-92 M8-6g×20-F:103
- Жесткий:115 [WeldJoint]: Крышка воды зад:1 ↔ Болт ГОСТ Р 50274-92 M8-6g×20-F:104
- Жесткий:116 [WeldJoint]: Крышка воды зад:1 ↔ Болт ГОСТ Р 50274-92 M8-6g×20-F:105
- Жесткий:117 [WeldJoint]: Крышка воды зад:1 ↔ Болт ГОСТ Р 50274-92 M8-6g×20-F:117
- Жесткий:118 [WeldJoint]: Крышка воды зад:1 ↔ Болт ГОСТ Р 50274-92 M8-6g×20-F:106
- Жесткий:119 [WeldJoint]: Крышка воды зад:1 ↔ Болт ГОСТ Р 50274-92 M8-6g×20-F:118
- Жесткий:120 [WeldJoint]: Крышка воды зад:1 ↔ Болт ГОСТ Р 50274-92 M8-6g×20-F:119
- Жесткий:121 [WeldJoint]: Крышка воды зад:1 ↔ Болт ГОСТ Р 50274-92 M8-6g×20-F:120
- Жесткий:122 [WeldJoint]: Крышка воды зад:1 ↔ Болт ГОСТ Р 50274-92 M8-6g×20-F:121
- Жесткий:123 [WeldJoint]: Крышка воды зад:1 ↔ Болт ГОСТ Р 50274-92 M8-6g×20-F:122
- Жесткий:124 [WeldJoint]: Крышка воды зад:1 ↔ Болт ГОСТ Р 50274-92 M8-6g×20-F:123
- Жесткий:125 [WeldJoint]: Крышка воды зад:1 ↔ Болт ГОСТ Р 50274-92 M8-6g×20-F:124
- Жесткий:126 [WeldJoint]: Крышка воды зад:1 ↔ Болт ГОСТ Р 50274-92 M8-6g×20-F:125
- Жесткий:127 [WeldJoint]: Крышка воды зад:1 ↔ Болт ГОСТ Р 50274-92 M8-6g×20-F:126
- Жесткий:128 [WeldJoint]: Крышка воды зад:1 ↔ Болт ГОСТ Р 50274-92 M8-6g×20-F:137
- Жесткий:129 [WeldJoint]: Крышка воды зад:1 ↔ Болт ГОСТ Р 50274-92 M8-6g×20-F:130
- Жесткий:130 [WeldJoint]: Крышка воды зад:1 ↔ Болт ГОСТ Р 50274-92 M8-6g×20-F:107
- Жесткий:131 [WeldJoint]: Крышка воды зад:1 ↔ Болт ГОСТ Р 50274-92 M8-6g×20-F:110
- Жесткий:132 [WeldJoint]: Крышка воды зад:1 ↔ Болт ГОСТ Р 50274-92 M8-6g×20-F:112
- Жесткий:133 [WeldJoint]: Крышка воды зад:1 ↔ Болт ГОСТ Р 50274-92 M8-6g×20-F:109
- Жесткий:134 [WeldJoint]: Крышка воды зад:1 ↔ Болт ГОСТ Р 50274-92 M8-6g×20-F:108
- Жесткий:135 [WeldJoint]: Крышка воды зад:1 ↔ Болт ГОСТ Р 50274-92 M8-6g×20-F:111
- Жесткий:136 [WeldJoint]: Крышка воды зад:1 ↔ Болт ГОСТ Р 50274-92 M8-6g×20-F:139
- Жесткий:137 [WeldJoint]: Крышка воды зад:1 ↔ Болт ГОСТ Р 50274-92 M8-6g×20-F:138
- Жесткий:138 [WeldJoint]: Крышка воды зад:1 ↔ Болт ГОСТ Р 50274-92 M8-6g×20-F:140
- Жесткий:139 [WeldJoint] (1 mm): Кольцо сальника:23 ↔ Пружина сальника:24
- Жесткий:140 [WeldJoint]: Кольцо сальника:22 ↔ Пружина сальника:23
- Жесткий:141 [WeldJoint]: Кольцо сальника:24 ↔ Пружина сальника:22
- Жесткий:142 [WeldJoint]: Крышка цилиндра 2:1 ↔ Шпилька ГОСТ 22034-76 M10-6g×45:1
- Жесткий:143 [WeldJoint]: Крышка сальников:1 ↔ Шайба ГОСТ 9065-75 12:1
- Жесткий:144 [WeldJoint]: Гайка ГОСТ 15521-70 M10:1 ↔ Шайба ГОСТ 9065-75 12:1
- Жесткий:145 [WeldJoint]: Крышка цилиндра 2:1 ↔ Фонарь:1
- С поворотом:16 [RevoluteJoint]: Крышка цилиндра 2:1 ↔ Шпилька ГОСТ 22038-76 M20-6g×80:1
- Жесткий:146 [WeldJoint]: Фонарь:1 ↔ Шайба ГОСТ 6402-70 22 L:1
- Жесткий:147 [WeldJoint]: Гайка ГОСТ ISO 8673-2014 M20x1,5:1 ↔ Шайба ГОСТ 6402-70 22 L:1
- Жесткий:148 [WeldJoint]: Кольцо сальника:25 ↔ Пружина сальника:25
- [WeldJoint]: Кольцо сальника:26 ↔ Пружина сальника:26
- [WeldJoint]: Кольцо сальника:27 ↔ Пружина сальника:27
- Жесткий:151 [WeldJoint]: Кольцо сальника:26 ↔ Кольцо сальника:27
- Жесткий:152 [WeldJoint]: Кольцо сальника:25 ↔ Кольцо сальника:27
- [WeldJoint]: Кольцо сальника:28 ↔ Пружина сальника:28
- [WeldJoint]: Кольцо сальника:29 ↔ Пружина сальника:29
- [WeldJoint]: Кольцо сальника:30 ↔ Пружина сальника:30
- [WeldJoint]: Кольцо сальника:29 ↔ Кольцо сальника:30
- [WeldJoint]: Кольцо сальника:28 ↔ Кольцо сальника:30
- Жесткий:158 [WeldJoint]: Корпус сальника перегородка 1:1 ↔ Кольцо сальника:26
- Жесткий:159 [WeldJoint]: Корпус сальника перегородка 1:1 ↔ Кольцо сальника:28
- Жесткий:160 [WeldJoint]: Фонарь:1 ↔ Крышка перегородки11:1
- Жесткий:161 [WeldJoint]: Корпус сальника перегородка 1:1 ↔ Крышка перегородки11:1
- Жесткий:162 [WeldJoint]: Корпус сальника перегородка 1:1 ↔ Крышка перегородки12:1
- Жесткий:163 [WeldJoint]: Крышка перегородки11:1 ↔ Придав перегородки1:1
- Жесткий:166 [WeldJoint]: Маслосъемное кольцо:1 ↔ Маслосъемное кольцо:2
- Жесткий:167 [WeldJoint]: Корпус маслосъемника:1 ↔ Маслосъемное кольцо:2
- Жесткий:168 [WeldJoint]: Фонарь:1 ↔ Крышка перегородки21:1
- [WeldJoint]: Кольцо сальника:31 ↔ Пружина сальника:31
- [WeldJoint]: Кольцо сальника:32 ↔ Пружина сальника:32
- [WeldJoint]: Кольцо сальника:33 ↔ Пружина сальника:33
- [WeldJoint]: Кольцо сальника:32 ↔ Кольцо сальника:33
- [WeldJoint]: Кольцо сальника:31 ↔ Кольцо сальника:33
- Жесткий:174 [WeldJoint]: Крышка перегородки21:1 ↔ Кольцо сальника:31
- Жесткий:175 [WeldJoint]: Корпус маслосъемника:1 ↔ Крышка перегородки21:1
- Жесткий:176 [WeldJoint]: Крышка перегородки21:1 ↔ Крышка перегородки22:1
- Жесткий:177 [WeldJoint]: Маслосъемное кольцо:1 ↔ Маслосъемная пружина:3
- Жесткий:178 [WeldJoint] (1 mm): Маслосъемное кольцо:2 ↔ Маслосъемная пружина:4
- Жесткий:179 [WeldJoint]: Крышка перегородки21:1 ↔ Придав перегородки1:2
- Жесткий:180 [WeldJoint]: Придав перегородки1:2 ↔ Шайба  ГОСТ 11371-78 13:1
- Жесткий:181 [WeldJoint]: Винт ГОСТ 11738-84 M 10x20:1 ↔ Шайба  ГОСТ 11371-78 13:1
- [WeldJoint]: Винт ГОСТ 11738-84 M 10x20:3 ↔ Шайба  ГОСТ 11371-78 13:3
- Жесткий:184 [WeldJoint]: Придав перегородки1:1 ↔ Шайба  ГОСТ 11371-78 13:3
- Жесткий:185 [WeldJoint]: Крышка перегородки22:1 ↔ Шайба  ГОСТ 11371-78 13:18
- Жесткий:186 [WeldJoint]: Шайба  ГОСТ 11371-78 13:18 ↔ Винт ГОСТ 11738-84 M 10x25:1
- [WeldJoint]: Винт ГОСТ 11738-84 M 10x25:2 ↔ Шайба  ГОСТ 11371-78 13:19
- Жесткий:188 [WeldJoint]: Крышка перегородки12:1 ↔ Шайба  ГОСТ 11371-78 13:19
- Жесткий:189 [WeldJoint]: Фонарь:1 ↔ Крейцкопфф:1
- [RevoluteJoint]: Верхняя часть поршня:2 ↔ Нижняя часть поршня:2
- [RevoluteJoint]: Верхняя часть поршня:2 ↔ Кольцо поршня:4
- [WeldJoint]: Нижняя часть поршня:2 ↔ Кольцо поршня:5
- [WeldJoint]: Нижняя часть поршня:2 ↔ Кольцо поршня:6
- [WeldJoint]: Верхняя часть поршня:2 ↔ Опорное кольцо:4
- [WeldJoint]: Нижняя часть поршня:2 ↔ Опорное кольцо:3
- [WeldJoint]: Кольцо поршень-шток низ:2 ↔ Нижняя часть поршня:2
- [WeldJoint]: Верхняя часть поршня:2 ↔ Кольцо поршень-шток верх:2
- [WeldJoint]: Гайка шток-поршень:2 ↔ Кольцо поршень-шток верх:2
- [WeldJoint]: Гайка шток-поршень:2 ↔ Шток:2
- Жесткий:198 [WeldJoint] (115 mm): Крышка цилиндра 1:1 ↔ Верхняя часть поршня:2
- Угол:1 [Angle] (45 deg): Крышка цилиндра 1:1 ↔ Крейцкопфф:1
- Угол:2 [Angle] (45 deg): Крышка цилиндра 1:1 ↔ Крейцкопфф:1
- Угол:3 [Angle] (45 deg): Крышка цилиндра 1:1 ↔ Крейцкопфф:1
- С поворотом:19 [RevoluteJoint]: Крейцкопфф:1 ↔ Вал:1
- Угол:4 [Angle] (0 deg): Крейцкопфф:1 ↔ Вал:1
- Заподлицо:9 [Flush]: Фонарь:1 ↔ Крышка фонаря 1:1
- Заподлицо:10 [Flush]: Фонарь:1 ↔ Крышка фонаря 1:1
- Заподлицо:11 [Flush]: Фонарь:1 ↔ Крышка фонаря 2:1
- Заподлицо:12 [Flush]: Фонарь:1 ↔ Крышка фонаря 2:1
- [Flush]: Картер:1 ↔ Крышка стенки картера низ:1
- [Flush]: Картер:1 ↔ Крышка стенки картера низ:1
- [WeldJoint]: Картер:1 ↔ Нижняя часть коренного подшипника:1
- [WeldJoint]: Картер:1 ↔ Нижняя часть коренного подшипника:2
- [Flush]: Картер:1 ↔ Крышка стенки картера верх:1
- [Flush]: Картер:1 ↔ Крышка стенки картера верх:1
- [WeldJoint]: Нижняя часть коренного подшипника:2 ↔ Нижняя часть коренного подшипника:4
- [WeldJoint]: Картер:1 ↔ Крышка коренного подшипника1:1
- [Flush]: Картер:1 ↔ Крышка картера 1:1
- [Flush]: Картер:1 ↔ Крышка картера 1:1
- [Flush]: Картер:1 ↔ Крышка картера 3:1
- [Flush]: Картер:1 ↔ Крышка картера 3:1
- [WeldJoint]: Картер:1 ↔ Балка:1
- [WeldJoint]: Картер:1 ↔ Балка:2
- [WeldJoint]: Картер:1 ↔ Крышка коренного подшипника1:2
- [WeldJoint]: Нижняя часть коренного подшипника:3 ↔ Крышка коренного подшипника1:2
- [WeldJoint]: Картер:1 ↔ Крышка стенки картера низ:1
- [WeldJoint]: Крышка стенки картера низ:1 ↔ Крышка стенки картера верх:1
- [WeldJoint]: Крышка стенки картера верх:1 ↔ Крышка картера 1:1
- [WeldJoint]: Картер:1 ↔ Крышка картера 3:1
- Жесткий:211 [WeldJoint]: Фонарь:1 ↔ Картер:1
- Цилиндрический:1 [CylindricalJoint]: Вал:1 ↔ Нижняя часть коренного подшипника:1
- Совмещение:1 [Mate] (5 mm): Вал:1 ↔ Крышка коренного подшипника1:2
## Named parameters: d45_d35 = -1 mm, d46_d36_d35 = -1 mm, d47_d37_d35 = -1 mm, d48_d38 = 0 mm, d49_d39 = 0 mm, d50_d40 = 0 mm, d53_d45_d35 = -1 mm, d54_d46_d36_d35 = -1 mm, d55_d47_d37_d35 = -1 mm, d56_d48_d38 = 0 mm, d57_d49_d39 = 0 mm, d58_d50_d40 = 0 mm, d60_d45_d35 = -1 mm, d61_d46_d36_d35 = -1 mm, d62_d47_d37_d35 = -1 mm, d63_d48_d38 = 0 mm, d64_d49_d39 = 0 mm, d65_d50_d40 = 0 mm, d67_d45_d35 = -1 mm, d68_d46_d36_d35 = -1 mm, d69_d47_d37_d35 = -1 mm, d70_d48_d38 = 0 mm, d71_d49_d39 = 0 mm, d72_d50_d40 = 0 mm, d74_d45_d35 = -1 mm, d75_d46_d36_d35 = -1 mm, d76_d47_d37_d35 = -1 mm, d77_d48_d38 = 0 mm, d78_d49_d39 = 0 mm, d79_d50_d40 = 0 mm, d81_d45_d35 = -1 mm, d82_d46_d36_d35 = -1 mm, d83_d47_d37_d35 = -1 mm, d84_d48_d38 = 0 mm, d85_d49_d39 = 0 mm, d86_d50_d40 = 0 mm, d101_d20 = 0 mm, d102_d21 = 30 deg, d114_d109 = 0 mm, d228_d227 = 0 mm, d229_d227 = 0 mm, d232_d227 = 0 mm, d233_d228_d227 = 0 mm, d234_d229_d227 = 0 mm, d235_d230 = 0 mm, d236_d231 = 0 mm, d248_d232_d227 = 0 mm, d249_d233_d228_d227 = 0 mm, d250_d234_d229_d227 = 0 mm, d251_d235_d230 = 0 mm, d252_d236_d231 = 0 mm, d262_d260 = 0 mm, d270_d269 = 0 mm, d278_d3 = 0 mm, d279_d4 = 105 deg, d280_d5 = 0 mm, d281_d6 = -75 deg, d282_d7 = 0 mm, d283_d8 = 0 mm, d284_d9 = 0 mm, d285_d10 = 0 mm, d286_d12 = 0 mm, d287_d20 = 0 mm, d288_d21 = 0 mm, d289_d22 = 0 mm, d10_d11 = 0 mm, d11_d13 = 0 mm, d310_d33 = 0 mm, d313_d23 = 0 mm, d314_d24 = 0 mm, d316_d28 = 0 mm, d317_d30 = 0 mm, d318_d31 = 0 mm, d319_d32 = 0 mm, d320_d42 = 0 mm, d321_d43 = 0 mm
